# Autodesk Inventor assembly: indexer
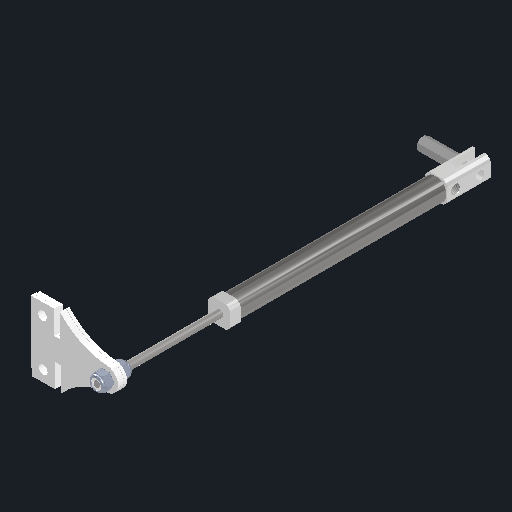
[picture p0: Inventor's stored thumbnail of the model, 512x512]
Saved by Autodesk Inventor 2023 (Build 270158000, 158)
## iProperties
Created: 2023-04-09
Part Number: indexer
Document SubType Name: Assembly
Designer: Windows Macbook
Author: Windows Macbook
## Documents named in this file (6)
- C:\Users\Windows Macbook\Desktop\VRC-SPIN-UP\Inventor\Assembly\Worlds\indexer.iam
- C:\Users\Windows Macbook\Desktop\VRC-SPIN-UP\Inventor\Structure\Hardware\Nut Nylock.ipt
- C:\Users\Windows Macbook\Desktop\VRC-SPIN-UP\Inventor\Assembly\Worlds\indexer.ipt
- C:\Users\Windows Macbook\Desktop\VRC-SPIN-UP\Inventor\Motion\Pneumatics\Single Acting Piston.iam
- C:\Users\Windows Macbook\Desktop\VRC-SPIN-UP\Inventor\Structure\Standoff\Standoff .75.ipt
- C:\Users\Windows Macbook\Desktop\VRC-SPIN-UP\Inventor\Structure\Standoff.ipt
## Components (7 placed, 4 different names)
1. Single Acting Piston:1 [sub-assembly] — Insert:1, Angle:1, Insert:8
2. Nut Nylock:1 — Insert:5
3. Nut Nylock:2 — Insert:1, Insert:2
4. indexer:1 — Insert:2, Insert:3, Insert:6, Angle:1
5. indexer:2 — Insert:4, Insert:5, Insert:7
6. indexer:3 — Insert:3, Insert:4, Insert:6, Insert:7
7. Standoff .75:1 — Insert:8
## Relationships (9: Insert 8, Angle 1)
- Insert:1 (10.16 mm): Single Acting Piston:1 ↔ Nut Nylock:2
- Insert:2: Nut Nylock:2 ↔ indexer:1
- Insert:3: indexer:1 ↔ indexer:3
- Insert:4: indexer:2 ↔ indexer:3
- Insert:5: Nut Nylock:1 ↔ indexer:2
- Insert:6: indexer:1 ↔ indexer:3
- Insert:7: indexer:2 ↔ indexer:3
- Angle:1 (0 deg): Single Acting Piston:1 ↔ indexer:1
- Insert:8: Single Acting Piston:1 ↔ Standoff .75:1
